# Autodesk Inventor assembly: ComederoV4
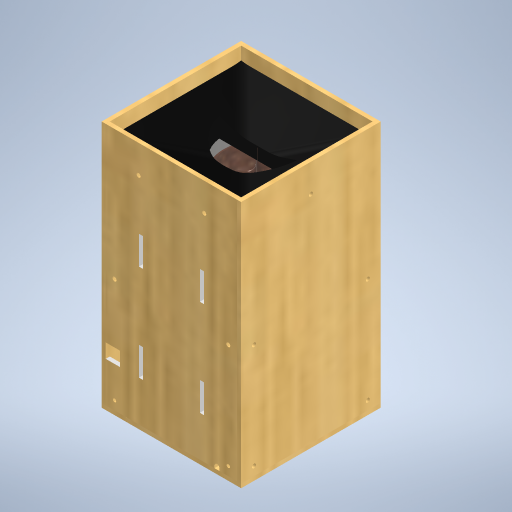
[picture p0: Inventor's stored thumbnail of the model, 512x512]
Saved by Autodesk Inventor 2024.2 (Build 282272000, 272)
## iProperties
Created: 2022-12-03
Part Number: ComederoV4
Document SubType Name: Assembly
Designer: sergi
Author: sergi
## Documents named in this file (21)
- C:\Users\sergi\OneDrive\Escritorio\Projects\Automatic Feeder\ComederoV4\Inventor\ComederoV4.iam
- C:\Users\sergi\OneDrive\Escritorio\Projects\Automatic Feeder\ComederoV4\Inventor\Panel1.ipt
- C:\Users\sergi\OneDrive\Escritorio\Projects\Automatic Feeder\ComederoV4\Inventor\Panel2.ipt
- C:\Users\sergi\OneDrive\Escritorio\Projects\Automatic Feeder\ComederoV4\Inventor\Panel3.ipt
- C:\Users\sergi\OneDrive\Escritorio\Projects\Automatic Feeder\ComederoV4\Inventor\Panel4.ipt
- C:\Users\sergi\OneDrive\Escritorio\Projects\Automatic Feeder\ComederoV4\Inventor\Embudo.ipt
- C:\Users\sergi\OneDrive\Escritorio\Projects\Automatic Feeder\ComederoV4\Inventor\Camisa.ipt
- C:\Users\sergi\OneDrive\Escritorio\Projects\Automatic Feeder\ComederoV4\Inventor\Madera intermedia.ipt
- C:\Users\sergi\OneDrive\Escritorio\Projects\Automatic Feeder\ComederoV4\Inventor\Tapa_abajo.ipt
- C:\Users\sergi\OneDrive\Escritorio\Projects\Automatic Feeder\ComederoV4\Inventor\Rampa2.ipt
- C:\Users\sergi\OneDrive\Escritorio\Projects\Automatic Feeder\ComederoV4\Inventor\Tambor2.ipt
- C:\Users\sergi\OneDrive\Escritorio\Projects\Automatic Feeder\ComederoV4\Inventor\motor_acople.iam
- C:\Users\sergi\OneDrive\Escritorio\Projects\Automatic Feeder\ComederoV4\Inventor\Soporte motor.ipt
- C:\Users\sergi\OneDrive\Escritorio\Projects\Automatic Feeder\ComederoV4\Inventor\Encoder.ipt
- C:\Users\sergi\OneDrive\Escritorio\Cuarto  Carrera\Mecatrónica\Caja conexiones\LCDmodule.ipt
- C:\Users\sergi\OneDrive\Escritorio\Projects\Automatic Feeder\ComederoV4\Inventor\Panel mando.ipt
- C:\Users\sergi\OneDrive\Escritorio\Projects\Automatic Feeder\ComederoV4\Inventor\Escuadra_triple.ipt
- C:\Users\sergi\OneDrive\Escritorio\Projects\Automatic Feeder\ComederoV4\Inventor\DriverCC.ipt
- C:\Users\sergi\OneDrive\Escritorio\Projects\Automatic Feeder\ComederoV4\Inventor\Arduino v5 (1).ipt
- C:\Users\sergi\OneDrive\Escritorio\Projects\Automatic Feeder\ComederoV4\Inventor\Tambor4.ipt
- C:\Users\sergi\OneDrive\Escritorio\Projects\Automatic Feeder\ComederoV4\Inventor\JHD162A\JHD162A.ipt
## Components (21 placed, 20 different names)
1. motor_acople:1 [sub-assembly] — Coincidencia:13, Coincidencia:14, Coincidencia:15, Coincidencia:45, Coincidencia:46
2. Panel1:1 — Coincidencia:1, Nivelación:1, Nivelación:2, Coincidencia:2, Nivelación:3, Nivelación:4, Coincidencia:9, Coincidencia:25, Nivelación:15, Coincidencia:26, Coincidencia:27, Coincidencia:28, Nivelación:16, Coincidencia:36, Coincidencia:38, Coincidencia:41
3. Panel2:1 — Coincidencia:1, Nivelación:1, Nivelación:2, Coincidencia:31, Coincidencia:33, Coincidencia:37, Coincidencia:39, Coincidencia:42, Coincidencia:43
4. Panel3:1 — Coincidencia:2, Nivelación:3, Nivelación:4, Nivelación:6, Nivelación:7, Coincidencia:3, Nivelación:8, Coincidencia:5, Coincidencia:6, Coincidencia:7, Coincidencia:8, Coincidencia:29
5. Panel4:1 — Nivelación:6, Nivelación:7, Coincidencia:3, Coincidencia:4, Nivelación:9, Coincidencia:30, Coincidencia:34
6. Rampa2:1 — Coincidencia:5, Coincidencia:6, Coincidencia:7, Coincidencia:10
7. Tambor2:1 — Coincidencia:20, Coincidencia:21
8. Tapa_abajo:1 — Coincidencia:4, Nivelación:8, Nivelación:9, Coincidencia:40
9. Madera intermedia:1 — Coincidencia:8, Coincidencia:9, Coincidencia:10, Coincidencia:11, Coincidencia:12, Coincidencia:17, Coincidencia:18, Coincidencia:19, Coincidencia:20, Coincidencia:32, Coincidencia:35, Ángulo:1
10. Soporte motor:1 — Coincidencia:11, Coincidencia:12, Coincidencia:13, Coincidencia:14, Coincidencia:15, Nivelación:11, Coincidencia:16, Nivelación:13, Ángulo:1
11. Encoder:1 — Nivelación:11, Coincidencia:16, Nivelación:13
12. Camisa:1 — Coincidencia:17, Coincidencia:18, Coincidencia:19, Coincidencia:21
13. Embudo:1 — Coincidencia:29, Coincidencia:30, Coincidencia:31, Coincidencia:44
14. LCDmodule:1 — Coincidencia:25, Nivelación:15, Coincidencia:26
15. Panel mando:1 — Coincidencia:27, Coincidencia:28, Nivelación:16
16. Escuadra_triple:1 — Coincidencia:32, Coincidencia:33, Coincidencia:34
17. Escuadra_triple:2 — Coincidencia:35, Coincidencia:36, Coincidencia:37
18. DriverCC:1 — Coincidencia:38, Coincidencia:39, Coincidencia:40
19. Arduino v5 (1):1 — Coincidencia:41, Coincidencia:42, Coincidencia:43
20. Tambor4:1 — Coincidencia:44, Coincidencia:45, Coincidencia:46
21. JHD162A:1
## Relationships (56: Mate 43, Flush 12, Angle 1)
- Coincidencia:1 [Mate]: Panel1:1 ↔ Panel2:1
- Nivelación:1 [Flush]: Panel1:1 ↔ Panel2:1
- Nivelación:2 [Flush]: Panel1:1 ↔ Panel2:1
- Coincidencia:2 [Mate]: Panel1:1 ↔ Panel3:1
- Nivelación:3 [Flush]: Panel1:1 ↔ Panel3:1
- Nivelación:4 [Flush]: Panel1:1 ↔ Panel3:1
- Nivelación:6 [Flush]: Panel3:1 ↔ Panel4:1
- Nivelación:7 [Flush]: Panel3:1 ↔ Panel4:1
- Coincidencia:3 [Mate]: Panel3:1 ↔ Panel4:1
- Coincidencia:4 [Mate]: Panel4:1 ↔ Tapa_abajo:1
- Nivelación:8 [Flush]: Panel3:1 ↔ Tapa_abajo:1
- Nivelación:9 [Flush]: Panel4:1 ↔ Tapa_abajo:1
- Coincidencia:5 [Mate]: Panel3:1 ↔ Rampa2:1
- Coincidencia:6 [Mate]: Panel3:1 ↔ Rampa2:1
- Coincidencia:7 [Mate]: Panel3:1 ↔ Rampa2:1
- Coincidencia:8 [Mate]: Panel3:1 ↔ Madera intermedia:1
- Coincidencia:9 [Mate]: Panel1:1 ↔ Madera intermedia:1
- Coincidencia:10 [Mate]: Rampa2:1 ↔ Madera intermedia:1
- Coincidencia:11 [Mate]: Madera intermedia:1 ↔ Soporte motor:1
- Coincidencia:12 [Mate]: Madera intermedia:1 ↔ Soporte motor:1
- Coincidencia:13 [Mate]: motor_acople:1 ↔ Soporte motor:1
- Coincidencia:14 [Mate]: motor_acople:1 ↔ Soporte motor:1
- Coincidencia:15 [Mate]: motor_acople:1 ↔ Soporte motor:1
- Nivelación:11 [Flush] (7 mm): Soporte motor:1 ↔ Encoder:1
- Coincidencia:16 [Mate]: Soporte motor:1 ↔ Encoder:1
- Nivelación:13 [Flush]: Soporte motor:1 ↔ Encoder:1
- Coincidencia:17 [Mate]: Madera intermedia:1 ↔ Camisa:1
- Coincidencia:18 [Mate]: Madera intermedia:1 ↔ Camisa:1
- Coincidencia:19 [Mate]: Madera intermedia:1 ↔ Camisa:1
- Coincidencia:20 [Mate]: Tambor2:1 ↔ Madera intermedia:1
- Coincidencia:21 [Mate]: Tambor2:1 ↔ Camisa:1
- Coincidencia:25 [Mate] (0.5 mm): Panel1:1 ↔ LCDmodule:1
- Nivelación:15 [Flush]: Panel1:1 ↔ LCDmodule:1
- Coincidencia:26 [Mate] (0.5 mm): Panel1:1 ↔ LCDmodule:1
- Coincidencia:27 [Mate] (1 mm): Panel1:1 ↔ Panel mando:1
- Coincidencia:28 [Mate] (1 mm): Panel1:1 ↔ Panel mando:1
- Nivelación:16 [Flush] (-5 mm): Panel1:1 ↔ Panel mando:1
- Coincidencia:29 [Mate]: Panel3:1 ↔ Embudo:1
- Coincidencia:30 [Mate]: Panel4:1 ↔ Embudo:1
- Coincidencia:31 [Mate]: Panel2:1 ↔ Embudo:1
- Coincidencia:32 [Mate]: Madera intermedia:1 ↔ Escuadra_triple:1
- Coincidencia:33 [Mate]: Panel2:1 ↔ Escuadra_triple:1
- Coincidencia:34 [Mate]: Panel4:1 ↔ Escuadra_triple:1
- Coincidencia:35 [Mate]: Madera intermedia:1 ↔ Escuadra_triple:2
- Coincidencia:36 [Mate]: Panel1:1 ↔ Escuadra_triple:2
- Coincidencia:37 [Mate]: Panel2:1 ↔ Escuadra_triple:2
- Ángulo:1 [Angle] (0 deg): Madera intermedia:1 ↔ Soporte motor:1
- Coincidencia:38 [Mate]: Panel1:1 ↔ DriverCC:1
- Coincidencia:39 [Mate] (60 mm): Panel2:1 ↔ DriverCC:1
- Coincidencia:40 [Mate] (20 mm): Tapa_abajo:1 ↔ DriverCC:1
- Coincidencia:41 [Mate]: Panel1:1 ↔ Arduino v5 (1):1
- Coincidencia:42 [Mate]: Panel2:1 ↔ Arduino v5 (1):1
- Coincidencia:43 [Mate] (10 mm): Panel2:1 ↔ Arduino v5 (1):1
- Coincidencia:44 [Mate]: Embudo:1 ↔ Tambor4:1
- Coincidencia:45 [Mate]: motor_acople:1 ↔ Tambor4:1
- Coincidencia:46 [Mate] (3 mm): motor_acople:1 ↔ Tambor4:1
